# Autodesk Inventor assembly: inhelationFilterHousing
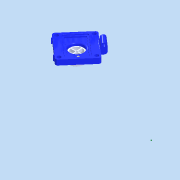
[picture p0: Inventor's stored thumbnail of the model, 180x180]
Saved by Autodesk Inventor 2020 (Build 240168000, 168)
## iProperties
Created: 2020-04-09
Part Number: inhelationFilterHousing
Document SubType Name: Assembly
Designer: Simon
Author: Simon
## Documents named in this file (3)
- D:\GrabCAD\MTL Ventilator Design\Filter housing with o ring\inhelationFilterHousing.iam
- D:\GrabCAD\MTL Ventilator Design\Filter housing with o ring\checkValve.ipt
- D:\GrabCAD\MTL Ventilator Design\Filter housing with o ring\filter housing for barb.ipt
## Components (2 placed, 2 different names)
1. checkValve:1 — Mate:1, Angle:1, Mate:2
2. filter housing for barb:1 — Mate:1, Angle:1, Mate:2
## Relationships (3: Mate 2, Angle 1)
- Mate:1: checkValve:1 ↔ filter housing for barb:1
- Angle:1 (45 deg): checkValve:1 ↔ filter housing for barb:1
- Mate:2: checkValve:1 ↔ filter housing for barb:1
